# Autodesk Inventor assembly: ASY NVPH-300 hopper
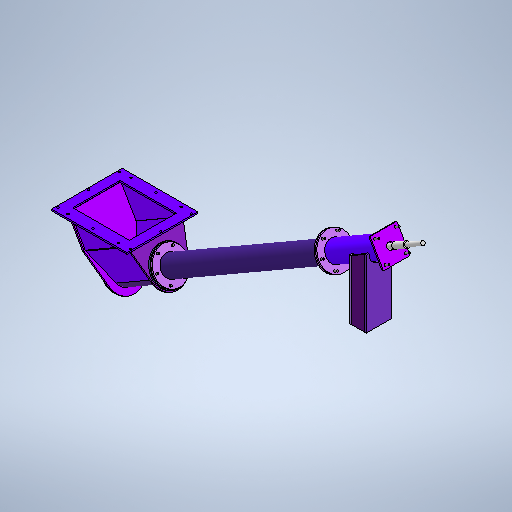
[picture p0: Inventor's stored thumbnail of the model, 512x512]
Saved by Autodesk Inventor 2025.1 (Build 291241020, 241B)
## iProperties
Created: 2024-12-19
Part Number: ASY NVPH-300 hopper
Document SubType Name: Assembly
Designer: admin
Author: admin
## Documents named in this file (10)
- C:\Users\user\YandexDisk-badmisterfox\home pc\Inventor\NDM-VOS_powder_hopper\ASY NVPH-300 hopper.iam
- C:\Users\user\YandexDisk-badmisterfox\home pc\Inventor\NDM-VOS_powder_hopper\ASY HPR 600 Feeder head.iam
- C:\Users\user\YandexDisk-badmisterfox\home pc\Inventor\NDM-VOS_powder_hopper\NVPH-307 right side.ipt
- C:\Users\user\YandexDisk-badmisterfox\home pc\Inventor\NDM-VOS_powder_hopper\NVPH-418 revision cup.ipt
- C:\Users\user\YandexDisk-badmisterfox\home pc\Inventor\NDM-VOS_powder_hopper\NVPH-324 conductor.ipt
- C:\Users\user\YandexDisk-badmisterfox\home pc\Inventor\NDM-VOS_powder_hopper\ASY HPR 340 hopper main tube.iam
- C:\Users\user\YandexDisk-badmisterfox\home pc\Inventor\NDM-VOS_powder_hopper\CC\en-US\ISO 4017(1)\ISO 4017 - M12 x 40 - ISO.ipt
- C:\Users\user\YandexDisk-badmisterfox\home pc\Inventor\NDM-VOS_powder_hopper\CC\en-US\ISO 4017(1)\ISO 4017 - M10 x 40 - ISO.ipt
- C:\Users\user\YandexDisk-badmisterfox\home pc\Inventor\NDM-VOS_powder_hopper\ASY HPR 320 hopper bin.iam
- C:\Users\user\YandexDisk-badmisterfox\home pc\Inventor\NDM-VOS_powder_hopper\ASY HPR 350 Auger.iam
## Components (18 placed, 9 different names)
1. ASY HPR 600 Feeder head:1 [sub-assembly] — Rotational:4, Rotational:10, Rotational:11, Rotational:12
2. NVPH-418 revision cup:1
3. NVPH-324 conductor:1
4. NVPH-324 conductor:2
5. ASY HPR 340 hopper main tube:1 [sub-assembly] — Rotational:5, Rotational:6, Rotational:7, Rotational:8, Rotational:3, Rotational:9
6. NVPH-307 right side:2
7. ISO 4017 M12 x 40:1 — Rotational:3
8. ISO 4017 M12 x 40:2 — Rotational:8
9. ISO 4017 M12 x 40:3 — Rotational:9
10. ISO 4017 M12 x 40:4 — Rotational:7
11. ISO 4017 M12 x 40:5 — Rotational:6
12. ISO 4017 M12 x 40:6 — Rotational:5
13. ISO 4017 M10 x 40:1 — Rotational:4
14. ISO 4017 M10 x 40:2 — Rotational:10
15. ISO 4017 M10 x 40:3 — Rotational:11
16. ISO 4017 M10 x 40:4 — Rotational:12
17. ASY HPR 320 hopper bin:1 [sub-assembly]
18. ASY HPR 350 Auger:1 [sub-assembly]
## Relationships (24: RevoluteJoint 10, WeldJoint 6, Mate 3, Flush 3, CylindricalJoint 2)
- [CylindricalJoint]: ASY HPR 340 hopper main tube:1 ↔ ASY HPR 350 Auger:1
- [CylindricalJoint]: ASY HPR 340 hopper main tube:1 ↔ ASY HPR 320 hopper bin:1
- [WeldJoint] (-2 mm): ASY HPR 600 Feeder head:1 ↔ ASY HPR 340 hopper main tube:1
- [WeldJoint]: NVPH-418 revision cup:1 ↔ ASY HPR 320 hopper bin:1
- [WeldJoint]: ASY HPR 340 hopper main tube:1 ↔ ASY HPR 320 hopper bin:1
- [WeldJoint]: ASY HPR 600 Feeder head:1 ↔ ASY HPR 340 hopper main tube:1
- [WeldJoint]: NVPH-324 conductor:2 ↔ ASY HPR 320 hopper bin:1
- [WeldJoint]: NVPH-324 conductor:1 ↔ ASY HPR 320 hopper bin:1
- [Mate]: ASY HPR 320 hopper bin:1
- [Mate]: ASY HPR 320 hopper bin:1
- [Flush]: ASY HPR 320 hopper bin:1
- [Mate]: ASY HPR 320 hopper bin:1
- [Flush]: ASY HPR 320 hopper bin:1
- Rotational:3 [RevoluteJoint]: ASY HPR 340 hopper main tube:1 ↔ ISO 4017 M12 x 40:1
- Rotational:4 [RevoluteJoint]: ASY HPR 600 Feeder head:1 ↔ ISO 4017 M10 x 40:1
- Rotational:5 [RevoluteJoint]: ASY HPR 340 hopper main tube:1 ↔ ISO 4017 M12 x 40:6
- Rotational:6 [RevoluteJoint]: ASY HPR 340 hopper main tube:1 ↔ ISO 4017 M12 x 40:5
- Rotational:7 [RevoluteJoint]: ASY HPR 340 hopper main tube:1 ↔ ISO 4017 M12 x 40:4
- Rotational:8 [RevoluteJoint]: ASY HPR 340 hopper main tube:1 ↔ ISO 4017 M12 x 40:2
- Rotational:9 [RevoluteJoint]: ASY HPR 340 hopper main tube:1 ↔ ISO 4017 M12 x 40:3
- Rotational:10 [RevoluteJoint]: ASY HPR 600 Feeder head:1 ↔ ISO 4017 M10 x 40:2
- Rotational:11 [RevoluteJoint]: ASY HPR 600 Feeder head:1 ↔ ISO 4017 M10 x 40:3
- Rotational:12 [RevoluteJoint]: ASY HPR 600 Feeder head:1 ↔ ISO 4017 M10 x 40:4
- [Flush] (241 mm): ASY HPR 600 Feeder head:1 ↔ ASY HPR 350 Auger:1
